# Autodesk Inventor assembly: recreat 3
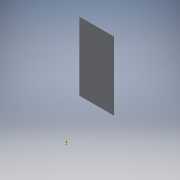
[picture p0: Inventor's stored thumbnail of the model, 180x180]
Saved by Autodesk Inventor 2019 (Build 230136000, 136)
## iProperties
Created: 2021-11-16
Part Number: recreat 3
Material: 一般
Document SubType Name: Assembly
Designer: yuta
Author: yuta
## Documents named in this file (6)
- C:\Users\yuta\Documents\キャチロボ\recreat 3.iam
- C:\Users\yuta\Documents\キャチロボ\NC.port.ipt
- C:\Users\yuta\Documents\キャチロボ\creat4.ipt
- C:\Users\yuta\Documents\キャチロボ\creat3.ipt
- C:\Users\yuta\Documents\キャチロボ\creat2.ipt
- C:\Users\yuta\Documents\キャチロボ\creat10.ipt
## Components (9 placed, 5 different names)
1. NC.port:1 — メイト:1, メイト:2, メイト:3, メイト:4, メイト:5
2. creat4:1 — メイト:1, メイト:2, メイト:6, メイト:7
3. creat4:2 — メイト:3, メイト:4, メイト:9, メイト:11
4. creat3:1 — メイト:5, メイト:6, メイト:8
5. creat3:2 — メイト:7, メイト:8, メイト:10
6. creat2:1 — メイト:9, メイト:10
7. creat10:2 — メイト:11
8. creat10:3
9. creat10:4
## Relationships (11: Mate 11)
- メイト:1 [Mate] (6 mm): NC.port:1 ↔ creat4:1
- メイト:2 [Mate] (6 mm): NC.port:1 ↔ creat4:1
- メイト:3 [Mate] (6 mm): NC.port:1 ↔ creat4:2
- メイト:4 [Mate] (6 mm): NC.port:1 ↔ creat4:2
- メイト:5 [Mate] (6 mm): NC.port:1 ↔ creat3:1
- メイト:6 [Mate] (6 mm): creat4:1 ↔ creat3:1
- メイト:7 [Mate] (6 mm): creat4:1 ↔ creat3:2
- メイト:8 [Mate] (6 mm): creat3:1 ↔ creat3:2
- メイト:9 [Mate] (6 mm): creat4:2 ↔ creat2:1
- メイト:10 [Mate] (6 mm): creat3:2 ↔ creat2:1
- メイト:11 [Mate] (6 mm): creat4:2 ↔ creat10:2
